# Autodesk Inventor assembly: z_assembly
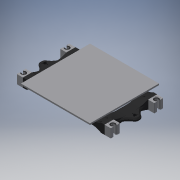
[picture p0: Inventor's stored thumbnail of the model, 180x180]
Saved by Autodesk Inventor 2017 (Build 210142000, 142)
## iProperties
Created: 2016-06-30
Part Number: z_assembly
Document SubType Name: Assembly
Designer: brent
Author: brent
## Documents named in this file (3)
- C:\Users\yibre\OneDrive\personal\printer_mechanical\z_assembly.iam
- C:\Users\yibre\OneDrive\personal\printer_mechanical\zaxis.ipt
- C:\Users\yibre\OneDrive\personal\printer_mechanical\offtheshelf\sbr12uu.ipt
## Components (5 placed, 2 different names)
1. zaxis:1 — Mate:9, Mate:10, Mate:11, Mate:12, Mate:13, Mate:14, Mate:15, Mate:16, Mate:17, Mate:18
2. sbr12uu:1 — Mate:17, Mate:18
3. sbr12uu:2 — Mate:14, Mate:15, Mate:16
4. sbr12uu:3 — Mate:11, Mate:12
5. sbr12uu:4 — Mate:9, Mate:10, Mate:13
## Relationships (10: Mate 10)
- Mate:9: zaxis:1 ↔ sbr12uu:4
- Mate:10: zaxis:1 ↔ sbr12uu:4
- Mate:11: zaxis:1 ↔ sbr12uu:3
- Mate:12: zaxis:1 ↔ sbr12uu:3
- Mate:13: zaxis:1 ↔ sbr12uu:4
- Mate:14: zaxis:1 ↔ sbr12uu:2
- Mate:15: zaxis:1 ↔ sbr12uu:2
- Mate:16: zaxis:1 ↔ sbr12uu:2
- Mate:17: zaxis:1 ↔ sbr12uu:1
- Mate:18: zaxis:1 ↔ sbr12uu:1
